# Autodesk Inventor assembly: CAttach1
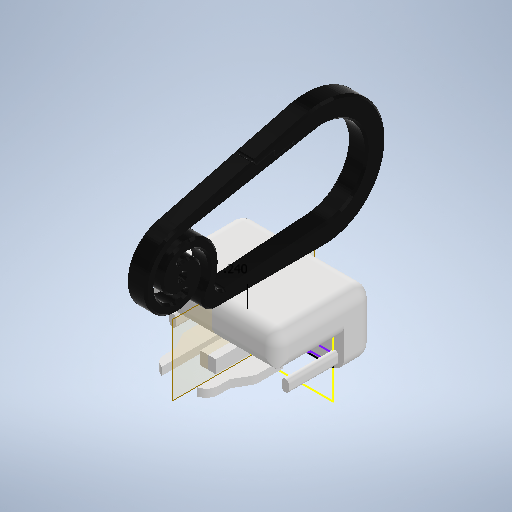
[picture p0: Inventor's stored thumbnail of the model, 512x512]
Saved by Autodesk Inventor 2025 (Build 290162010, 162A)
## iProperties
Created: 2026-05-19
Part Number: CAttach1
Document SubType Name: Assembly
Designer: 925699
Author: 925699
## Documents named in this file (3)
- C:\Users\925699\Documents\Inventor\Spirabiner\CAttach1.iam
- C:\Users\925699\Documents\Inventor\Spirabiner\Attachment11S.ipt
- C:\Users\925699\Documents\Inventor\Spirabiner\Part1.ipt
## Components (2 placed, 2 different names)
1. Attachment11S:1 — Rigid:1
2. Part1:1 — Rigid:1
## Relationships (1: WeldJoint 1)
- Rigid:1 [WeldJoint]: Attachment11S:1 ↔ Part1:1
